# Autodesk Inventor assembly: Assembly2
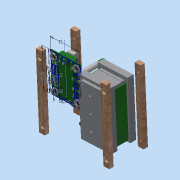
[picture p0: Inventor's stored thumbnail of the model, 180x180]
Saved by Autodesk Inventor 2015 (Build 190159000, 159)
## iProperties
Created: 2015-01-31
Part Number: Assembly2
Document SubType Name: Assembly
Designer: Openlab
Author: Openlab
## Documents named in this file (14)
- C:\Users\Openlab\Documents\Alexey\HS-Spectrophotometer\parts\Assembly2.iam
- C:\Users\Openlab\Documents\Alexey\HS-Spectrophotometer\parts\Bottom.ipt
- C:\Users\Openlab\Documents\Alexey\HS-Spectrophotometer\parts\Base_V3.ipt
- C:\Users\Openlab\Documents\Alexey\HS-Spectrophotometer\parts\Top_V3.ipt
- C:\Users\Openlab\Documents\Alexey\HS-Spectrophotometer\parts\Led_Board_V1.ipt
- C:\Users\Openlab\Documents\Alexey\HS-Spectrophotometer\parts\Sensor_Board_dummy.ipt
- C:\Users\Openlab\Documents\Alexey\HS-Spectrophotometer\parts\Top_plate.ipt
- C:\Users\Openlab\Documents\Alexey\HS-Spectrophotometer\parts\Front_wall.ipt
- C:\Users\Openlab\Documents\Alexey\HS-Spectrophotometer\parts\Bask_Wall.ipt
- C:\Users\Openlab\Documents\Alexey\HS-Spectrophotometer\parts\Rail.ipt
- C:\Users\Openlab\Documents\Alexey\HS-Spectrophotometer\parts\Motherboard_dummy.ipt
- C:\Users\Openlab\Documents\Alexey\HS-Spectrophotometer\parts\Support_washer.ipt
- C:\Users\Openlab\Documents\Alexey\HS-Spectrophotometer\parts\Left_wall.ipt
- C:\Users\Openlab\Documents\Alexey\HS-Spectrophotometer\parts\Right_wall.ipt
## Components (19 placed, 13 different names)
1. Bottom:1 — Mate:3, Mate:4, Mate:5, Mate:12, Mate:13, Mate:14, Mate:33, Mate:34, Mate:35, Mate:36, Mate:37, Mate:38, Mate:39, Mate:40, Mate:41, Mate:42, Mate:43, Mate:44, Mate:45, Mate:46, Mate:49, Mate:53, Mate:56, Mate:57
2. Base_V3:1 — Mate:1, Mate:2, Flush:1, Mate:3, Mate:4, Mate:5, Mate:6, Mate:7, Mate:9, Mate:11, Mate:50
3. Top_V3:1 — Mate:1, Mate:2, Flush:1, Mate:8
4. Led_Board_V1:1 — Mate:9, Mate:11, Mate:50
5. Sensor_Board_dummy:1 — Mate:6, Mate:7, Mate:8
6. Top_plate:1 — Mate:15, Mate:16, Mate:17, Mate:24, Mate:26, Mate:27, Mate:28, Mate:29, Mate:30, Mate:31, Mate:32, Mate:54
7. Front_wall:1 — Mate:12, Mate:13, Mate:14, Mate:15, Mate:16, Mate:17, Mate:52
8. Bask_Wall:1 — Mate:24, Mate:26, Mate:51, Mate:55
9. Rail:1 — Mate:27, Mate:30, Mate:32
10. Rail:2 — Mate:28, Mate:29, Mate:31
11. Rail:3 — Mate:34, Mate:35, Mate:36
12. Rail:4 — Mate:33, Mate:37, Mate:38
13. Motherboard_dummy:1 — Mate:47, Mate:48, Mate:49
14. Support_washer:1 — Mate:39, Mate:43
15. Support_washer:2 — Mate:40, Mate:44, Mate:47
16. Support_washer:3 — Mate:42, Mate:46, Mate:48
17. Support_washer:4 — Mate:41, Mate:45
18. Left_wall:1 — Mate:51, Mate:52, Mate:53, Mate:57
19. Right_wall:1 — Mate:54, Mate:55, Mate:56
## Relationships (50: Mate 49, Flush 1)
- Mate:1: Base_V3:1 ↔ Top_V3:1
- Mate:2: Base_V3:1 ↔ Top_V3:1
- Flush:1: Base_V3:1 ↔ Top_V3:1
- Mate:3: Bottom:1 ↔ Base_V3:1
- Mate:4: Bottom:1 ↔ Base_V3:1
- Mate:5: Bottom:1 ↔ Base_V3:1
- Mate:6: Base_V3:1 ↔ Sensor_Board_dummy:1
- Mate:7: Base_V3:1 ↔ Sensor_Board_dummy:1
- Mate:8: Top_V3:1 ↔ Sensor_Board_dummy:1
- Mate:9: Base_V3:1 ↔ Led_Board_V1:1
- Mate:11: Base_V3:1 ↔ Led_Board_V1:1
- Mate:12: Bottom:1 ↔ Front_wall:1
- Mate:13: Bottom:1 ↔ Front_wall:1
- Mate:14: Bottom:1 ↔ Front_wall:1
- Mate:15: Top_plate:1 ↔ Front_wall:1
- Mate:16: Top_plate:1 ↔ Front_wall:1
- Mate:17: Top_plate:1 ↔ Front_wall:1
- Mate:24: Top_plate:1 ↔ Bask_Wall:1
- Mate:26: Top_plate:1 ↔ Bask_Wall:1
- Mate:27: Top_plate:1 ↔ Rail:1
- Mate:28: Top_plate:1 ↔ Rail:2
- Mate:29: Top_plate:1 ↔ Rail:2
- Mate:30: Top_plate:1 ↔ Rail:1
- Mate:31: Top_plate:1 ↔ Rail:2
- Mate:32: Top_plate:1 ↔ Rail:1
- Mate:33: Bottom:1 ↔ Rail:4
- Mate:34: Bottom:1 ↔ Rail:3
- Mate:35: Bottom:1 ↔ Rail:3
- Mate:36: Bottom:1 ↔ Rail:3
- Mate:37: Bottom:1 ↔ Rail:4
- Mate:38: Bottom:1 ↔ Rail:4
- Mate:39: Bottom:1 ↔ Support_washer:1
- Mate:40: Bottom:1 ↔ Support_washer:2
- Mate:41: Bottom:1 ↔ Support_washer:4
- Mate:42: Bottom:1 ↔ Support_washer:3
- Mate:43: Bottom:1 ↔ Support_washer:1
- Mate:44: Bottom:1 ↔ Support_washer:2
- Mate:45: Bottom:1 ↔ Support_washer:4
- Mate:46: Bottom:1 ↔ Support_washer:3
- Mate:47: Motherboard_dummy:1 ↔ Support_washer:2
- Mate:48: Motherboard_dummy:1 ↔ Support_washer:3
- Mate:49: Bottom:1 ↔ Motherboard_dummy:1
- Mate:50: Base_V3:1 ↔ Led_Board_V1:1
- Mate:51: Bask_Wall:1 ↔ Left_wall:1
- Mate:52: Front_wall:1 ↔ Left_wall:1
- Mate:53: Bottom:1 ↔ Left_wall:1
- Mate:54: Top_plate:1 ↔ Right_wall:1
- Mate:55: Bask_Wall:1 ↔ Right_wall:1
- Mate:56: Bottom:1 ↔ Right_wall:1
- Mate:57: Bottom:1 ↔ Left_wall:1
